# Autodesk Inventor assembly: ASY MSC 900.7 base frame transverse
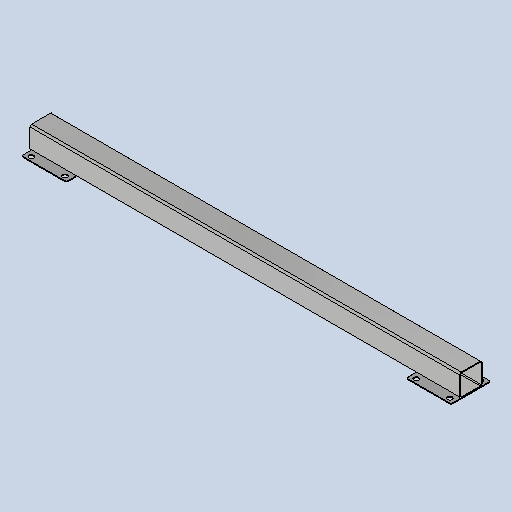
[picture p0: Inventor's stored thumbnail of the model, 512x512]
Saved by Autodesk Inventor 2025 (Build 290162010, 162A)
## iProperties
Created: 2024-09-07
Part Number: ASY MSC 900.7 base frame transverse
Document SubType Name: Assembly
Designer: pokla
Author: pokla
## Documents named in this file (3)
- C:\Users\admin\YandexDisk-badmisterfox\домашниий пк\Inventor\Manturovo\Manturovo_Se-clar\ASY MSC 900.7 base frame transverse.iam
- C:\Users\admin\YandexDisk-badmisterfox\домашниий пк\Inventor\Manturovo\Manturovo_Se-clar\MSC 908 transverse pillar plate.ipt
- C:\Users\admin\YandexDisk-badmisterfox\домашниий пк\Inventor\Manturovo\Manturovo_Se-clar\ISO 4019 - 80x80x3 - 2925.ipt
## Components (3 placed, 2 different names)
1. MSC 908 transverse pillar plate.ipt:1
2. MSC 908 transverse pillar plate.ipt:2 — Rigid:2
3. ISO 4019 - 80x80x3 - 2925.ipt:1 — Rigid:2
## Relationships (2: WeldJoint 2)
- [WeldJoint]: MSC 908 transverse pillar plate.ipt:1 ↔ ISO 4019 - 80x80x3 - 2925.ipt:1
- Rigid:2 [WeldJoint]: MSC 908 transverse pillar plate.ipt:2 ↔ ISO 4019 - 80x80x3 - 2925.ipt:1
